# Autodesk Inventor assembly: 200-50-WHEEL-CONNECTOR-30MM-ASM-01
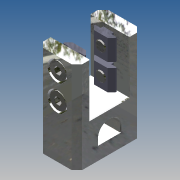
[picture p0: Inventor's stored thumbnail of the model, 180x180]
Saved by Autodesk Inventor 2018.2 (Build 222227000, 227)
## iProperties
Manager: feesmrt
Company: FRANC0R
Created: 2017-12-18
Part Number: 200-50-WHEEL-CONNECTOR-30MM-ASM-01
Document SubType Name: Assembly
Designer: feesmrt
Project: Rescue Robot
Cost Center: -
Description: Wheel Connector 30mm - ASM
Engineer: feesmrt
Authority: feesmrt
Stock Number: 200-50-WHEEL-CONNECTOR-30MM-ASM-01
Author: feesmrt
Title: Wheel Connector 30mm - ASM
Subject: Rescue Robot
Revision Number: 1
## Documents named in this file (6)
- D:\Programmierung\FRANC0R\CAD\02-Rocker-Bogie-Robot\200-ROCKER-BOGIE\200-50-WHEEL-CONNECTOR\200-50-WHEEL-CONNECTOR-30MM-ASM-01.iam
- D:\Programmierung\FRANC0R\CAD\02-Rocker-Bogie-Robot\200-ROCKER-BOGIE\200-50-WHEEL-CONNECTOR\200-50-WHEEL-CONNECTOR-30MM-01.ipt
- D:\Programmierung\FRANC0R\CAD\02-Rocker-Bogie-Robot\200-ROCKER-BOGIE\200-50-WHEEL-CONNECTOR\200-50-WHEEL-CONNECTOR-30MM-02.ipt
- D:\Programmierung\FRANC0R\CAD\02-Rocker-Bogie-Robot\900-COMPONENTS\900-40-SCREWS\900-40-SCREWS-DIN7984_M5x10.ipt
- D:\Programmierung\FRANC0R\CAD\02-Rocker-Bogie-Robot\900-COMPONENTS\900-50-PROFILES\900-50-PROFILES-CONN-N8xM8.ipt
- D:\Programmierung\FRANC0R\CAD\02-Rocker-Bogie-Robot\900-COMPONENTS\900-40-SCREWS\900-40-SCREWS-DIN7984_M8x12.ipt
## Components (12 placed, 5 different names)
1. 200-50-WHEEL-CONNECTOR-30MM-01:1 — Passend:3, Passend:4, Passend:5, Passend:10, Passend:11, Passend:12, Passend:13, Winkel:1, Winkel:2, Passend:14, Passend:15, Passend:16, Passend:17, Winkel:3, Winkel:4, Passend:18, Passend:19, Passend:20, Passend:21, Passend:22, Passend:23, Passend:24, Passend:25
2. 200-50-WHEEL-CONNECTOR-30MM-02:1 — Passend:3, Passend:4, Passend:5, Passend:6, Passend:7, Passend:8, Passend:9
3. 900-40-SCREWS-DIN7984_M5x10:1 — Passend:6, Passend:9
4. 900-40-SCREWS-DIN7984_M5x10:2 — Passend:7, Passend:8
5. 900-50-PROFILES-CONN-N8xM8:1 — Passend:10, Passend:13, Winkel:1
6. 900-50-PROFILES-CONN-N8xM8:2 — Passend:11, Passend:12, Winkel:2
7. 900-50-PROFILES-CONN-N8xM8:3 — Passend:14, Passend:16, Winkel:3
8. 900-50-PROFILES-CONN-N8xM8:4 — Passend:15, Passend:17, Winkel:4
9. 900-40-SCREWS-DIN7984_M8x12:1 — Passend:18, Passend:24
10. 900-40-SCREWS-DIN7984_M8x12:2 — Passend:19, Passend:25
11. 900-40-SCREWS-DIN7984_M8x12:3 — Passend:20, Passend:23
12. 900-40-SCREWS-DIN7984_M8x12:4 — Passend:21, Passend:22
## Relationships (27: Mate 23, Angle 4)
- Passend:3 [Mate]: 200-50-WHEEL-CONNECTOR-30MM-01:1 ↔ 200-50-WHEEL-CONNECTOR-30MM-02:1
- Passend:4 [Mate]: 200-50-WHEEL-CONNECTOR-30MM-01:1 ↔ 200-50-WHEEL-CONNECTOR-30MM-02:1
- Passend:5 [Mate]: 200-50-WHEEL-CONNECTOR-30MM-01:1 ↔ 200-50-WHEEL-CONNECTOR-30MM-02:1
- Passend:6 [Mate]: 200-50-WHEEL-CONNECTOR-30MM-02:1 ↔ 900-40-SCREWS-DIN7984_M5x10:1
- Passend:7 [Mate]: 200-50-WHEEL-CONNECTOR-30MM-02:1 ↔ 900-40-SCREWS-DIN7984_M5x10:2
- Passend:8 [Mate]: 200-50-WHEEL-CONNECTOR-30MM-02:1 ↔ 900-40-SCREWS-DIN7984_M5x10:2
- Passend:9 [Mate]: 200-50-WHEEL-CONNECTOR-30MM-02:1 ↔ 900-40-SCREWS-DIN7984_M5x10:1
- Passend:10 [Mate]: 200-50-WHEEL-CONNECTOR-30MM-01:1 ↔ 900-50-PROFILES-CONN-N8xM8:1
- Passend:11 [Mate]: 200-50-WHEEL-CONNECTOR-30MM-01:1 ↔ 900-50-PROFILES-CONN-N8xM8:2
- Passend:12 [Mate] (2.8 mm): 200-50-WHEEL-CONNECTOR-30MM-01:1 ↔ 900-50-PROFILES-CONN-N8xM8:2
- Passend:13 [Mate] (2.8 mm): 200-50-WHEEL-CONNECTOR-30MM-01:1 ↔ 900-50-PROFILES-CONN-N8xM8:1
- Winkel:1 [Angle] (0 deg): 200-50-WHEEL-CONNECTOR-30MM-01:1 ↔ 900-50-PROFILES-CONN-N8xM8:1
- Winkel:2 [Angle] (0 deg): 200-50-WHEEL-CONNECTOR-30MM-01:1 ↔ 900-50-PROFILES-CONN-N8xM8:2
- Passend:14 [Mate]: 200-50-WHEEL-CONNECTOR-30MM-01:1 ↔ 900-50-PROFILES-CONN-N8xM8:3
- Passend:15 [Mate]: 200-50-WHEEL-CONNECTOR-30MM-01:1 ↔ 900-50-PROFILES-CONN-N8xM8:4
- Passend:16 [Mate] (2.8 mm): 200-50-WHEEL-CONNECTOR-30MM-01:1 ↔ 900-50-PROFILES-CONN-N8xM8:3
- Passend:17 [Mate] (2.8 mm): 200-50-WHEEL-CONNECTOR-30MM-01:1 ↔ 900-50-PROFILES-CONN-N8xM8:4
- Winkel:3 [Angle] (0 deg): 200-50-WHEEL-CONNECTOR-30MM-01:1 ↔ 900-50-PROFILES-CONN-N8xM8:3
- Winkel:4 [Angle] (0 deg): 200-50-WHEEL-CONNECTOR-30MM-01:1 ↔ 900-50-PROFILES-CONN-N8xM8:4
- Passend:18 [Mate]: 200-50-WHEEL-CONNECTOR-30MM-01:1 ↔ 900-40-SCREWS-DIN7984_M8x12:1
- Passend:19 [Mate]: 200-50-WHEEL-CONNECTOR-30MM-01:1 ↔ 900-40-SCREWS-DIN7984_M8x12:2
- Passend:20 [Mate]: 200-50-WHEEL-CONNECTOR-30MM-01:1 ↔ 900-40-SCREWS-DIN7984_M8x12:3
- Passend:21 [Mate]: 200-50-WHEEL-CONNECTOR-30MM-01:1 ↔ 900-40-SCREWS-DIN7984_M8x12:4
- Passend:22 [Mate]: 200-50-WHEEL-CONNECTOR-30MM-01:1 ↔ 900-40-SCREWS-DIN7984_M8x12:4
- Passend:23 [Mate]: 200-50-WHEEL-CONNECTOR-30MM-01:1 ↔ 900-40-SCREWS-DIN7984_M8x12:3
- Passend:24 [Mate]: 200-50-WHEEL-CONNECTOR-30MM-01:1 ↔ 900-40-SCREWS-DIN7984_M8x12:1
- Passend:25 [Mate]: 200-50-WHEEL-CONNECTOR-30MM-01:1 ↔ 900-40-SCREWS-DIN7984_M8x12:2
